# Autodesk Inventor assembly: Tetrix_739083
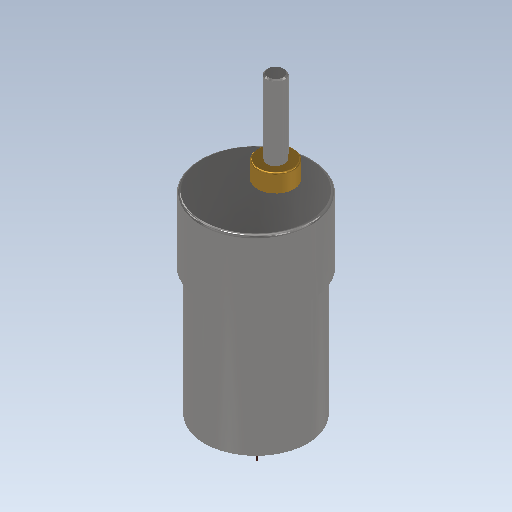
[picture p0: Inventor's stored thumbnail of the model, 512x512]
Saved by Autodesk Inventor 2020 (Build 240168000, 168)
## iProperties
Created: 2014-11-19
Part Number: Tetrix_739083
Document SubType Name: Assembly
Designer: Tetrix
Catalog Web Link: http://www.tetrixrobotics.com/TETRIX_DC_Gear_Motor
Vendor: Tetrix
Category: Motors
Company: Autodesk Inc.
Author: Autodesk Inc.
## Documents named in this file (3)
- D:\Documents\GitHub\AO_Robotics\CAD\Parts Kits\FTC Tetrix KOP Organized (7-24-19)\Motor\Tetrix_39083.iam
- D:\Documents\GitHub\AO_Robotics\CAD\Parts Kits\FTC Tetrix KOP Organized (7-24-19)\Motor\Assembly Components\Tetrix_39083_Motor.ipt
- D:\Documents\GitHub\AO_Robotics\CAD\Parts Kits\FTC Tetrix KOP Organized (7-24-19)\Motor\Assembly Components\Tetrix_39083_Axle.ipt
## Components (2 placed, 2 different names)
1. Tetrix_739083_Motor — Insert:1
2. Tetrix_739083_Axle — Insert:1
## Relationships (1: Insert 1)
- Insert:1: Tetrix_739083_Motor ↔ Tetrix_739083_Axle
